# Autodesk Inventor assembly: Butterfly Drive Base
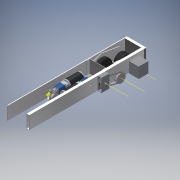
[picture p0: Inventor's stored thumbnail of the model, 180x180]
Saved by Autodesk Inventor 2019 (Build 230136000, 136)
## iProperties
Created: 2019-10-19
Part Number: Butterfly Drive Base
Document SubType Name: Assembly
Designer: Mark
Author: Mark
## Documents named in this file (16)
- C:\Users\Mark\Desktop\7738 Helion Engineering\7738-CAD-prep\Butterfly drive\Butterfly Drive Base.iam
- C:\Users\Mark\Desktop\7738 Helion Engineering\7738-CAD-prep\Butterfly drive\Butterfly Drive Module.iam
- C:\Users\Mark\Desktop\7738 Helion Engineering\7738-CAD-prep\Butterfly drive\Side Extrusion.ipt
- C:\Users\Mark\Desktop\7738 Helion Engineering\7738-CAD-prep\Butterfly drive\Module Plate 1.ipt
- C:\Users\Mark\Desktop\7738 Helion Engineering\7738-CAD-prep\Butterfly drive\Back Extrusion 1.ipt
- C:\Users\Mark\Desktop\7738 Helion Engineering\7738-CAD-prep\Butterfly drive\Bumper Plate.ipt
- C:\Users\Mark\Desktop\7738 Helion Engineering\7738-CAD-prep\Butterfly drive\Side Front Extrusion.ipt
- C:\Users\Mark\Desktop\7738 Helion Engineering\7738-CAD-prep\Butterfly drive\F6800Z 10mm ID Flange.ipt
- C:\Users\Mark\Desktop\7738 Helion Engineering\7738-CAD-prep\2 Stage HD - CIM Sport.iam
- C:\Users\Mark\Desktop\7738 Helion Engineering\7738-CAD-prep\am-0255 2.5inch CIM Motor.ipt
- C:\Users\Mark\Desktop\7738 Helion Engineering\7738-CAD-prep\Butterfly drive\Spacer Extrusion.ipt
- C:\Users\Mark\Desktop\7738 Helion Engineering\7738-CAD-prep\Butterfly drive\Butterfly Drive Base\Design Accelerator\Bevel Gears2.iam
- C:\Users\Mark\Desktop\7738 Helion Engineering\7738-CAD-prep\Butterfly drive\Motor Protection Extrusion.ipt
- C:\Users\Mark\Desktop\7738 Helion Engineering\7738-CAD-prep\Butterfly drive\Butterfly Drive Base\Design Accelerator\Synchronous Belts Transmission3.iam
- C:\Users\Mark\Desktop\7738 Helion Engineering\7738-CAD-prep\transmition Axle Support.ipt
- C:\Users\Mark\Desktop\7738 Helion Engineering\7738-CAD-prep\Butterfly drive\SDA 63 50.ipt
## Components (22 placed, 14 different names)
1. Butterfly Drive Module:1 [sub-assembly] — Angle:1, Mate:8, Mate:11, Mate:13, Mate:28
2. Side Extrusion:1 — Mate:1, Flush:1, Angle:1, Flush:7, Mate:10, Flush:8, Mate:12, Mate:14, Flush:9, Mate:20, Mate:26, Symmetry:1, Flush:10, Mate:29, Angle:2, Flush:11, Mate:36, Flush:12, Flush:15, Angle:3, Mate:45, Mate:46, Mate:47, Flush:18
3. Back Extrusion 1:1 — Mate:1, Flush:1, Mate:6, Flush:4, Flush:5, Mate:7, Flush:6
4. Bumper Plate:1 — Flush:5, Mate:7, Mate:8, Flush:6, Mate:26, Mate:28, Mate:35, Mate:37, Flush:13, Mate:57
5. Side Front Extrusion:1 — Flush:7, Mate:10, Flush:8, Symmetry:1, Mate:30, Mate:51
6. F6800Z 10mm ID Flange:1 — Mate:11, Mate:12
7. F6800Z 10mm ID Flange:2 — Mate:13, Mate:14
8. 2 Stage HD - CIM Sport:1 [sub-assembly] — Mate:15, Mate:16, Mate:17, Mate:20, Mate:33, Mate:34, Flush:15, Flush:16, Mate:51, Mate:54, Mate:55, Mate:56
9. am-0255 2.5inch CIM Motor:1 — Mate:15, Mate:16, Mate:17, Flush:17
10. 2 Stage HD - CIM Sport:2 [sub-assembly] — Mate:32, Flush:16, Mate:41, Flush:17, Mate:57
11. am-0255 2.5inch CIM Motor:2
12. Spacer Extrusion:2 — Flush:10, Mate:29, Mate:30
13. Bevel Gears:2 [sub-assembly] — Mate:33, Angle:2, Mate:34, Mate:43
14. Bevel Gears:3 [sub-assembly] — Mate:32, Mate:41
15. Spacer Extrusion:3 — Flush:11, Mate:35
16. Motor Protection Extrusion:1 — Mate:36, Flush:12
17. Motor Protection Extrusion:2 — Mate:37, Flush:13
18. Synchronous Belts Transmission:1 [sub-assembly] — Mate:48, Mate:53
19. F6800Z 10mm ID Flange:3 — Mate:45, Mate:46
20. transmition Axle Support:1 — Mate:47, Flush:18, Mate:48, Mate:49, Mate:50, Mate:53
21. F6800Z 10mm ID Flange:4 — Mate:49, Mate:50, Mate:52
22. SDA 63 50:1
## Relationships (60: Mate 41, Flush 15, Angle 3, Symmetry 1)
- Mate:1: Side Extrusion:1 ↔ Back Extrusion 1:1
- Flush:1: Side Extrusion:1 ↔ Back Extrusion 1:1
- Mate:6: Back Extrusion 1:1
- Flush:4: Back Extrusion 1:1
- Angle:1 (10 deg): Butterfly Drive Module:1 ↔ Side Extrusion:1
- Flush:5: Back Extrusion 1:1 ↔ Bumper Plate:1
- Mate:7: Back Extrusion 1:1 ↔ Bumper Plate:1
- Mate:8: Butterfly Drive Module:1 ↔ Bumper Plate:1
- Flush:6: Back Extrusion 1:1 ↔ Bumper Plate:1
- Flush:7: Side Extrusion:1 ↔ Side Front Extrusion:1
- Mate:10: Side Extrusion:1 ↔ Side Front Extrusion:1
- Flush:8: Side Extrusion:1 ↔ Side Front Extrusion:1
- Mate:11: Butterfly Drive Module:1 ↔ F6800Z 10mm ID Flange:1
- Mate:12 (0.3 mm): Side Extrusion:1 ↔ F6800Z 10mm ID Flange:1
- Mate:13: Butterfly Drive Module:1 ↔ F6800Z 10mm ID Flange:2
- Mate:14 (0.3 mm): Side Extrusion:1 ↔ F6800Z 10mm ID Flange:2
- Flush:9 (-18.548 mm): Side Extrusion:1
- Mate:15: 2 Stage HD - CIM Sport:1 ↔ am-0255 2.5inch CIM Motor:1
- Mate:16: 2 Stage HD - CIM Sport:1 ↔ am-0255 2.5inch CIM Motor:1
- Mate:17 (0.6 mm): 2 Stage HD - CIM Sport:1 ↔ am-0255 2.5inch CIM Motor:1
- Mate:20 (0.6 mm): Side Extrusion:1 ↔ 2 Stage HD - CIM Sport:1
- [Mate]: 2 Stage HD - CIM Sport:2 ↔ am-0255 2.5inch CIM Motor:2
- [Mate]: 2 Stage HD - CIM Sport:2 ↔ am-0255 2.5inch CIM Motor:2
- [Mate] (0.6 mm): 2 Stage HD - CIM Sport:2 ↔ am-0255 2.5inch CIM Motor:2
- Mate:26 (126 mm): Side Extrusion:1 ↔ Bumper Plate:1
- Symmetry:1: Side Extrusion:1 ↔ Side Front Extrusion:1
- Mate:28 (0.3 mm): Butterfly Drive Module:1 ↔ Bumper Plate:1
- Flush:10: Side Extrusion:1 ↔ Spacer Extrusion:2
- Mate:29 (0.5 mm): Side Extrusion:1 ↔ Spacer Extrusion:2
- Mate:30 (270 mm): Side Front Extrusion:1 ↔ Spacer Extrusion:2
- Mate:32: 2 Stage HD - CIM Sport:2 ↔ Bevel Gears:3
- Mate:33: 2 Stage HD - CIM Sport:1 ↔ Bevel Gears:2
- Angle:2 (180 deg): Side Extrusion:1 ↔ Bevel Gears:2
- Mate:34 (2 mm): 2 Stage HD - CIM Sport:1 ↔ Bevel Gears:2
- Flush:11: Side Extrusion:1 ↔ Spacer Extrusion:3
- Mate:35: Bumper Plate:1 ↔ Spacer Extrusion:3
- Mate:36 (0.5 mm): Side Extrusion:1 ↔ Motor Protection Extrusion:1
- Flush:12: Side Extrusion:1 ↔ Motor Protection Extrusion:1
- Mate:37 (0.5 mm): Bumper Plate:1 ↔ Motor Protection Extrusion:2
- Flush:13: Bumper Plate:1 ↔ Motor Protection Extrusion:2
- Flush:15 (26.1875 mm): Side Extrusion:1 ↔ 2 Stage HD - CIM Sport:1
- Flush:16: 2 Stage HD - CIM Sport:1 ↔ 2 Stage HD - CIM Sport:2
- Mate:41 (2 mm): 2 Stage HD - CIM Sport:2 ↔ Bevel Gears:3
- Mate:43: Bevel Gears:2
- Angle:3 (0 deg): Side Extrusion:1
- Flush:17: am-0255 2.5inch CIM Motor:1 ↔ 2 Stage HD - CIM Sport:2
- Mate:45: Side Extrusion:1 ↔ F6800Z 10mm ID Flange:3
- Mate:46 (0.3 mm): Side Extrusion:1 ↔ F6800Z 10mm ID Flange:3
- Mate:47 (0.6 mm): Side Extrusion:1 ↔ transmition Axle Support:1
- Flush:18: Side Extrusion:1 ↔ transmition Axle Support:1
- Mate:48 (-30 mm): Synchronous Belts Transmission:1 ↔ transmition Axle Support:1
- Mate:49: transmition Axle Support:1 ↔ F6800Z 10mm ID Flange:4
- Mate:50 (0.3 mm): transmition Axle Support:1 ↔ F6800Z 10mm ID Flange:4
- Mate:51 (374.508 mm): Side Front Extrusion:1 ↔ 2 Stage HD - CIM Sport:1
- Mate:52: F6800Z 10mm ID Flange:4
- Mate:53 (5 mm): Synchronous Belts Transmission:1 ↔ transmition Axle Support:1
- Mate:54: 2 Stage HD - CIM Sport:1
- Mate:55: 2 Stage HD - CIM Sport:1
- Mate:56: 2 Stage HD - CIM Sport:1
- Mate:57 (13.375 mm): Bumper Plate:1 ↔ 2 Stage HD - CIM Sport:2
## Named parameters: Height = 70 mm, ExtSta = 1 deg, ModuleAngle = 10 deg, d58_d50 = 0.6 mm, d59_d48 = 0 mm, d60_d49 = 0 mm
